# Autodesk Inventor assembly: 276-2010
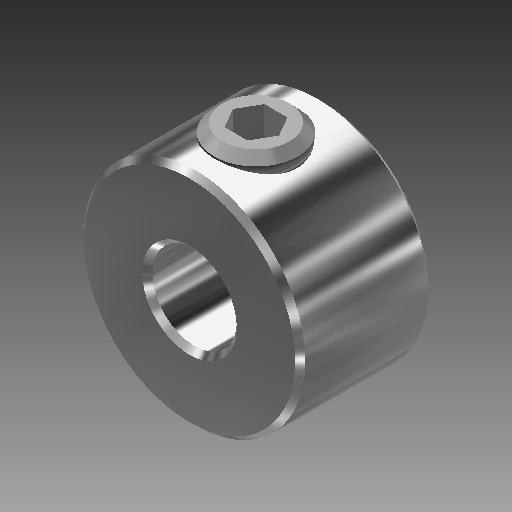
[picture p0: Inventor's stored thumbnail of the model, 512x512]
Saved by Autodesk Inventor 2018 (Build 220112000, 112)
## iProperties
Company: Autodesk Inc.
Category: Motion
Created: 2012-04-11
Document SubType Name: Assembly
Designer: Autodesk Inc.
Part Number: 276-2010
Catalog Web Link: http://www.vexrobotics.com/276-2010.html
Vendor: VEX
Author: Autodesk Inc.
## Documents named in this file (3)
- C:\Users\USER\Downloads\Inventor_2013_VEX_ KOP_-_Metric\Metric\Motion\Shaft Collar.iam
- C:\Users\USER\Downloads\Inventor_2013_VEX_ KOP_-_Metric\Metric\Motion\Components\Shaft Collar.ipt
- C:\Users\USER\Downloads\Inventor_2013_VEX_ KOP_-_Metric\Metric\Motion\Components\ANSI B18.3 - 8-32 UNC - 0.1875(32)306.ipt
## Components (2 placed, 2 different names)
1. Shaft Collar:1 — Mate:1, Flush:1, Angle:1
2. Type B - Hexagon Socket Set Screw - Cup Point - Inch 8-32 UNC - 0.1875:1 — Mate:1, Flush:1, Angle:1
## Relationships (3: Mate 1, Flush 1, Angle 1)
- Mate:1: Shaft Collar:1 ↔ Type B - Hexagon Socket Set Screw - Cup Point - Inch 8-32 UNC - 0.1875:1
- Flush:1 (-0.508 mm): Shaft Collar:1 ↔ Type B - Hexagon Socket Set Screw - Cup Point - Inch 8-32 UNC - 0.1875:1
- Angle:1 (0 deg): Shaft Collar:1 ↔ Type B - Hexagon Socket Set Screw - Cup Point - Inch 8-32 UNC - 0.1875:1
